# Autodesk Inventor assembly: Case
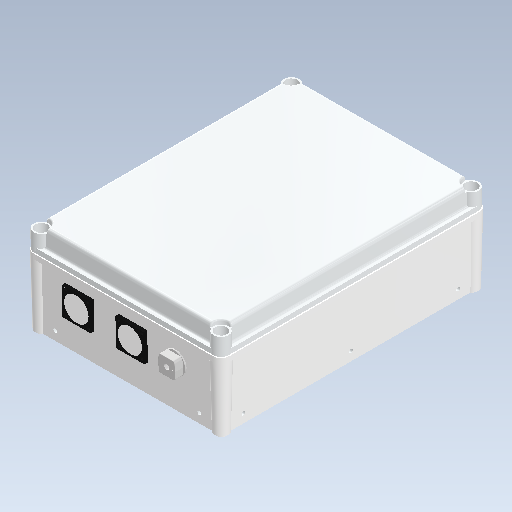
[picture p0: Inventor's stored thumbnail of the model, 512x512]
Saved by Autodesk Inventor 2020 (Build 240168000, 168)
## iProperties
Created: 2019-12-11
Part Number: Case
Document SubType Name: Assembly
Designer: nicoc
Author: nicoc
## Documents named in this file (13)
- D:\Repos\P5-AIonFPGA\cad\Case\Case.iam
- D:\Repos\P5-AIonFPGA\cad\Case\Ultra96\PWB_USDEV1-1_FINAL.iam
- D:\Repos\P5-AIonFPGA\cad\Case\Terminalblock\Terminalblock.iam
- D:\Repos\P5-AIonFPGA\cad\Case\SlottedWiring\SlottexWiring200mm.ipt
- D:\Repos\P5-AIonFPGA\cad\Case\SlottedWiring\SlottexWiring110mm.ipt
- D:\Repos\P5-AIonFPGA\cad\Case\Fibox_PC_3828 _3_T_Bottom.ipt
- D:\Repos\P5-AIonFPGA\cad\Case\Fibox_PC_3828 _3_T_Top.ipt
- D:\Repos\P5-AIonFPGA\cad\Case\Ventilator\Fan_40x40x20.iam
- D:\Repos\P5-AIonFPGA\cad\Case\Ventilator\Fan_60x60x25.ipt
- D:\Repos\P5-AIonFPGA\cad\Case\Ultra96\USBCable.ipt
- D:\Repos\P5-AIonFPGA\cad\Case\Ventilator\Filter40x40.ipt
- D:\Repos\P5-AIonFPGA\cad\Case\QuickCableGlandes\QuickCableGlandes.ipt
- D:\Repos\P5-AIonFPGA\cad\Case\Ventilator\Filter60x60.ipt
## Components (19 placed, 12 different names)
1. PWB_USDEV1-1_FINAL:1 [sub-assembly] — Mate:4, Mate:5, Mate:8, Mate:23, Flush:20, Flush:21
2. Terminalblock:1 [sub-assembly] — Mate:6, Mate:7
3. SlottexWiring200mm:1 — Mate:2, Flush:2, Flush:3, Flush:4
4. SlottexWiring200mm:2 — Mate:1, Flush:1, Flush:4, Mate:7, Mate:8
5. SlottexWiring110mm:1 — Mate:1, Flush:1, Mate:2, Flush:2, Flush:3, Mate:3, Mate:5
6. Fibox_PC_3828 _3_T_Bottom:1 — Mate:3, Mate:4, Mate:6, Mate:21, Mate:24, Mate:25, Mate:27, Tangent:2, Mate:28, Mate:29, Mate:30, Tangent:3, Tangent:4, Tangent:5, Mate:31, Mate:32
7. Fibox_PC_3828 _3_T_Top:1 — Mate:21
8. Fan_40x40x20:1 [sub-assembly] — Flush:24, Flush:25
9. Fan_40x40x20:3 [sub-assembly] — Flush:22, Flush:23
10. Fan_60x60x25:1 — Flush:27, Flush:28
11. USBCable:1 — Mate:23, Flush:20, Flush:21
12. Filter40x40:1 — Mate:25, Flush:24, Flush:25, Flush:26
13. Filter40x40:2 — Mate:24, Flush:22, Flush:23, Flush:26
14. QuickCableGlandes:1 — Mate:27, Tangent:2
15. QuickCableGlandes:2 — Mate:28, Tangent:4
16. QuickCableGlandes:3 — Mate:29, Tangent:5
17. QuickCableGlandes:4 — Mate:30, Tangent:3
18. Filter60x60:1 — Mate:32
19. Filter60x60:2 — Mate:31, Flush:27, Flush:28
## Relationships (35: Mate 18, Flush 13, Tangent 4)
- Mate:1: SlottexWiring200mm:2 ↔ SlottexWiring110mm:1
- Flush:1: SlottexWiring200mm:2 ↔ SlottexWiring110mm:1
- Mate:2: SlottexWiring200mm:1 ↔ SlottexWiring110mm:1
- Flush:2: SlottexWiring200mm:1 ↔ SlottexWiring110mm:1
- Flush:3: SlottexWiring200mm:1 ↔ SlottexWiring110mm:1
- Flush:4: SlottexWiring200mm:1 ↔ SlottexWiring200mm:2
- Mate:3: SlottexWiring110mm:1 ↔ Fibox_PC_3828 _3_T_Bottom:1
- Mate:4: PWB_USDEV1-1_FINAL:1 ↔ Fibox_PC_3828 _3_T_Bottom:1
- Mate:5 (40 mm): PWB_USDEV1-1_FINAL:1 ↔ SlottexWiring110mm:1
- Mate:6: Terminalblock:1 ↔ Fibox_PC_3828 _3_T_Bottom:1
- Mate:7 (10 mm): Terminalblock:1 ↔ SlottexWiring200mm:2
- Mate:8 (12.5 mm): PWB_USDEV1-1_FINAL:1 ↔ SlottexWiring200mm:2
- Mate:21: Fibox_PC_3828 _3_T_Bottom:1 ↔ Fibox_PC_3828 _3_T_Top:1
- Mate:23: PWB_USDEV1-1_FINAL:1 ↔ USBCable:1
- Flush:20: PWB_USDEV1-1_FINAL:1 ↔ USBCable:1
- Flush:21 (1 mm): PWB_USDEV1-1_FINAL:1 ↔ USBCable:1
- Mate:24: Fibox_PC_3828 _3_T_Bottom:1 ↔ Filter40x40:2
- Flush:22: Fan_40x40x20:3 ↔ Filter40x40:2
- Flush:23: Fan_40x40x20:3 ↔ Filter40x40:2
- Mate:25: Fibox_PC_3828 _3_T_Bottom:1 ↔ Filter40x40:1
- Flush:24: Fan_40x40x20:1 ↔ Filter40x40:1
- Flush:25: Fan_40x40x20:1 ↔ Filter40x40:1
- Flush:26: Filter40x40:1 ↔ Filter40x40:2
- Mate:27: Fibox_PC_3828 _3_T_Bottom:1 ↔ QuickCableGlandes:1
- Tangent:2: Fibox_PC_3828 _3_T_Bottom:1 ↔ QuickCableGlandes:1
- Mate:28: Fibox_PC_3828 _3_T_Bottom:1 ↔ QuickCableGlandes:2
- Mate:29: Fibox_PC_3828 _3_T_Bottom:1 ↔ QuickCableGlandes:3
- Mate:30: Fibox_PC_3828 _3_T_Bottom:1 ↔ QuickCableGlandes:4
- Tangent:3: Fibox_PC_3828 _3_T_Bottom:1 ↔ QuickCableGlandes:4
- Tangent:4: Fibox_PC_3828 _3_T_Bottom:1 ↔ QuickCableGlandes:2
- Tangent:5: Fibox_PC_3828 _3_T_Bottom:1 ↔ QuickCableGlandes:3
- Mate:31: Fibox_PC_3828 _3_T_Bottom:1 ↔ Filter60x60:2
- Mate:32: Fibox_PC_3828 _3_T_Bottom:1 ↔ Filter60x60:1
- Flush:27: Fan_60x60x25:1 ↔ Filter60x60:2
- Flush:28: Fan_60x60x25:1 ↔ Filter60x60:2
